# Autodesk Inventor assembly: PLA_SetCollar_d6_穴付き
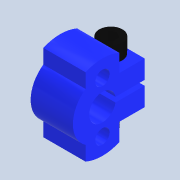
[picture p0: Inventor's stored thumbnail of the model, 180x180]
Saved by Autodesk Inventor 2021.2 (Build 252289000, 289)
## iProperties
Created: 2020-12-13
Part Number: PLA_SetCollar_d6_穴付き
Document SubType Name: Assembly
Designer: Hagihara Yuya
Author: Hagihara Yuya
## Documents named in this file (4)
- C:\Users\Hagihara Yuya\Documents\GrabCAD\NHK2021\BasicParts\よく使う部品（萩原）\SetColor\PLA_SetCollar_d6\PLA_SetCollar_d6_穴付き.iam
- C:\Users\Hagihara Yuya\Documents\GrabCAD\NHK2021\BasicParts\よく使う部品（萩原）\SetColor\PLA_SetCollar_d6\PLA_SetColor_d6_穴付き.ipt
- C:\Users\Hagihara Yuya\Documents\GrabCAD\NHK2021\BasicParts\よく使う部品（萩原）\SetColor\PLA_SetCollar_d6\Bolt_M3_15_for_SetCollar_d6.ipt
- C:\Users\Hagihara Yuya\Documents\GrabCAD\NHK2021\BasicParts\よく使う部品（萩原）\SetColor\PLA_SetCollar_d6\Nut_M3_for_SetCollar.ipt
## Components (3 placed, 3 different names)
1. PLA_SetColor_d6_穴付き:1 — 回転:1, 回転:2
2. Bolt_M3_15_for_SetCollar_d6:1 — 回転:1
3. Nut_M3_for_SetCollar:1 — 回転:2
## Relationships (2: RevoluteJoint 2)
- 回転:1 [RevoluteJoint]: PLA_SetColor_d6_穴付き:1 ↔ Bolt_M3_15_for_SetCollar_d6:1
- 回転:2 [RevoluteJoint]: PLA_SetColor_d6_穴付き:1 ↔ Nut_M3_for_SetCollar:1
